# Autodesk Inventor assembly: Assembly
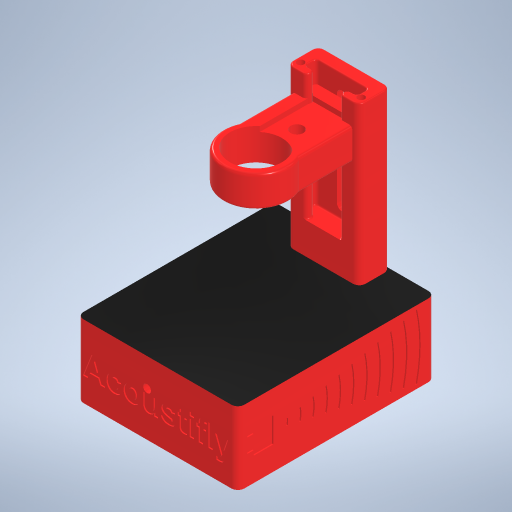
[picture p0: Inventor's stored thumbnail of the model, 512x512]
Saved by Autodesk Inventor 2023.3 (Build 273359000, 359)
## iProperties
Created: 2024-05-30
Part Number: Assembly
Document SubType Name: Assembly
Designer: Sven
Author: Sven
## Documents named in this file (8)
- C:\Users\Sven\Documents\Gitlab\Acoustifly\CAD\1_Col_Print\Assembly.iam
- C:\Users\Sven\Documents\Gitlab\Acoustifly\CAD\1_Col_Print\3D-PrintedParts\Base.ipt
- C:\Users\Sven\Documents\Gitlab\Acoustifly\CAD\1_Col_Print\OtherParts\MainPCB_Acoustifly.ipt
- C:\Users\Sven\Documents\Gitlab\Acoustifly\CAD\1_Col_Print\3D-PrintedParts\VerticalProfile.ipt
- C:\Users\Sven\Documents\Gitlab\Acoustifly\CAD\1_Col_Print\OtherParts\Transducer16mm.ipt
- C:\Users\Sven\Documents\Gitlab\Acoustifly\CAD\1_Col_Print\OtherParts\TransducerPCB_Acoustifly.ipt
- C:\Users\Sven\Documents\Gitlab\Acoustifly\CAD\1_Col_Print\3D-PrintedParts\TransducerPCB_Holder.ipt
- C:\Users\Sven\Documents\Gitlab\Acoustifly\CAD\1_Col_Print\3D-PrintedParts\Battery_Cover.ipt
## Components (7 placed, 7 different names)
1. Base:1 — Mate:1, Mate:2, Angle:1, Flush:1, Mate:3, Angle:2, Angle:3, Flush:3
2. MainPCB_Acoustifly:1 — Mate:1, Mate:2, Angle:1
3. VerticalProfile:1 — Flush:1
4. Transducer16mm:1 — Mate:3, Mate:4, Angle:2, Mate:5, Mate:6
5. TransducerPCB_Acoustifly:1 — Mate:5, Mate:6, Angle:3, Flush:2
6. TransducerPCB_Holder:1 — Flush:2
7. Battery_Cover:1 — Flush:3
## Relationships (12: Mate 6, Angle 3, Flush 3)
- Mate:1: Base:1 ↔ MainPCB_Acoustifly:1
- Mate:2: Base:1 ↔ MainPCB_Acoustifly:1
- Angle:1 (180 deg): Base:1 ↔ MainPCB_Acoustifly:1
- Flush:1: Base:1 ↔ VerticalProfile:1
- Mate:3 (30.1 mm): Base:1 ↔ Transducer16mm:1
- Mate:4: Transducer16mm:1
- Angle:2 (0 deg): Base:1 ↔ Transducer16mm:1
- Mate:5 (0.75 mm): Transducer16mm:1 ↔ TransducerPCB_Acoustifly:1
- Mate:6: Transducer16mm:1 ↔ TransducerPCB_Acoustifly:1
- Angle:3 (0 deg): Base:1 ↔ TransducerPCB_Acoustifly:1
- Flush:2: TransducerPCB_Acoustifly:1 ↔ TransducerPCB_Holder:1
- Flush:3: Base:1 ↔ Battery_Cover:1
